# Autodesk Inventor assembly: 000 Ensamblaje hw_LM - BASIC
(part 2 of 3)
- Flush:121: RES-1.6K_1%_0402:40 ↔ RES-1.6K_1%_0402:43
- Mate:81: hw_LM - PCB:1 ↔ C1206C152KGRACAUTO:1
- Flush:122: C1206C152KGRACAUTO:3 ↔ C1206C152KGRACAUTO:4
- Flush:123: C1206C152KGRACAUTO:2 ↔ C1206C152KGRACAUTO:3
- Flush:124: C1206C152KGRACAUTO:1 ↔ C1206C152KGRACAUTO:2
- Flush:125: BLM21PG220SN1D:12 ↔ BLM21PG220SN1D:13
- Flush:126: BLM21PG220SN1D:13 ↔ BLM21PG220SN1D:14
- Flush:127: BLM21PG220SN1D:14 ↔ BLM21PG220SN1D:15
- [Flush]: AQ24CANFD-02HTG:6 ↔ AQ24CANFD-02HTG:7
- [Flush]: AQ24CANFD-02HTG:7 ↔ AQ24CANFD-02HTG:8
- [Flush]: AQ24CANFD-02HTG:5 ↔ AQ24CANFD-02HTG:8
- Mate:83: hw_LM - PCB:1 ↔ HX5008NL:3
- Flush:137: RES-1.6K_1%_0402:55 ↔ RES-1.6K_1%_0402:59
- Flush:138: RES-1.6K_1%_0402:44 ↔ RES-1.6K_1%_0402:56
- Flush:139: RES-1.6K_1%_0402:52 ↔ RES-1.6K_1%_0402:59
- Flush:142: RES-1.6K_1%_0402:23 ↔ RES-1.6K_1%_0402:47
- Mate:84: hw_LM - PCB:1 ↔ RES-1.6K_1%_0402:56
- Flush:143: RES-1.6K_1%_0402:48 ↔ RES-1.6K_1%_0402:57
- Flush:144: RES-1.6K_1%_0402:56 ↔ RES-1.6K_1%_0402:57
- Flush:145: RES-1.6K_1%_0402:55 ↔ RES-1.6K_1%_0402:59
- Flush:146: RES-1.6K_1%_0402:56 ↔ RES-1.6K_1%_0402:58
- Flush:147: RES-1.6K_1%_0402:55 ↔ RES-1.6K_1%_0402:59
- Flush:148: RES-1.6K_1%_0402:52 ↔ RES-1.6K_1%_0402:53
- Flush:149: RES-1.6K_1%_0402:54 ↔ RES-1.6K_1%_0402:55
- Flush:150: RES-1.6K_1%_0402:55 ↔ RES-1.6K_1%_0402:59
- Flush:151: RES-1.6K_1%_0402:56 ↔ RES-1.6K_1%_0402:59
- Flush:152: RES-1.6K_1%_0402:49 ↔ RES-1.6K_1%_0402:52
- Flush:153: RES-1.6K_1%_0402:50 ↔ RES-1.6K_1%_0402:51
- Flush:154: RES-1.6K_1%_0402:51 ↔ RES-1.6K_1%_0402:55
- Flush:155: RES-1.6K_1%_0402:44 ↔ RES-1.6K_1%_0402:46
- Flush:156: RES-1.6K_1%_0402:45 ↔ RES-1.6K_1%_0402:55
- [Flush]: RES-1.6K_1%_0402:60 ↔ RES-1.6K_1%_0402:62
- Flush:158: RES-1.6K_1%_0402:47 ↔ RES-1.6K_1%_0402:63
- Flush:159: RES-1.6K_1%_0402:60 ↔ RES-1.6K_1%_0402:63
- Flush:160: RES-1.6K_1%_0402:61 ↔ RES-1.6K_1%_0402:63
- [Flush]: RES-1.6K_1%_0402:64 ↔ RES-1.6K_1%_0402:66
- [Flush]: RES-1.6K_1%_0402:64 ↔ RES-1.6K_1%_0402:67
- [Flush]: RES-1.6K_1%_0402:65 ↔ RES-1.6K_1%_0402:67
- Flush:164: RES-1.6K_1%_0402:62 ↔ RES-1.6K_1%_0402:65
- [Flush]: RES-1.6K_1%_0402:68 ↔ RES-1.6K_1%_0402:70
- [Flush]: RES-1.6K_1%_0402:68 ↔ RES-1.6K_1%_0402:71
- [Flush]: RES-1.6K_1%_0402:69 ↔ RES-1.6K_1%_0402:71
- Flush:168: RES-1.6K_1%_0402:62 ↔ RES-1.6K_1%_0402:69
- [Flush]: RES-1.6K_1%_0402:72 ↔ RES-1.6K_1%_0402:73
- [Flush]: RES-1.6K_1%_0402:72 ↔ RES-1.6K_1%_0402:73
- [Flush]: RES-1.6K_1%_0402:74 ↔ RES-1.6K_1%_0402:75
- [Flush]: RES-1.6K_1%_0402:74 ↔ RES-1.6K_1%_0402:75
- [Flush]: RES-1.6K_1%_0402:73 ↔ RES-1.6K_1%_0402:74
- Flush:174: RES-1.6K_1%_0402:72 ↔ RES-1.6K_1%_0402:75
- Flush:175: RES-1.6K_1%_0402:63 ↔ RES-1.6K_1%_0402:74
- [Flush]: RES-1.6K_1%_0402:76 ↔ RES-1.6K_1%_0402:77
- [Flush]: RES-1.6K_1%_0402:76 ↔ RES-1.6K_1%_0402:77
- [Flush]: RES-1.6K_1%_0402:78 ↔ RES-1.6K_1%_0402:79
- [Flush]: RES-1.6K_1%_0402:78 ↔ RES-1.6K_1%_0402:79
- [Flush]: RES-1.6K_1%_0402:77 ↔ RES-1.6K_1%_0402:78
- [Flush]: RES-1.6K_1%_0402:76 ↔ RES-1.6K_1%_0402:79
- Flush:182: RES-1.6K_1%_0402:67 ↔ RES-1.6K_1%_0402:79
- Flush:183: RES-1.6K_1%_0402:66 ↔ RES-1.6K_1%_0402:76
- [Flush]: RES-1.6K_1%_0402:80 ↔ RES-1.6K_1%_0402:81
- [Flush]: RES-1.6K_1%_0402:80 ↔ RES-1.6K_1%_0402:81
- Flush:186: RES-1.6K_1%_0402:78 ↔ RES-1.6K_1%_0402:80
- [Flush]: RES-1.6K_1%_0402:82 ↔ RES-1.6K_1%_0402:83
- [Flush]: RES-1.6K_1%_0402:82 ↔ RES-1.6K_1%_0402:84
- [Flush]: RES-1.6K_1%_0402:84 ↔ RES-1.6K_1%_0402:85
- Flush:190: RES-1.6K_1%_0402:82 ↔ RES-1.6K_1%_0402:83
- Flush:191: RES-1.6K_1%_0402:83 ↔ RES-1.6K_1%_0402:84
- Flush:192: RES-1.6K_1%_0402:84 ↔ RES-1.6K_1%_0402:85
- Flush:194: RES-1.6K_1%_0402:85 ↔ RES-1.6K_1%_0402:86
- [Flush]: RES-1.6K_1%_0402:87 ↔ RES-1.6K_1%_0402:88
- [Flush]: RES-1.6K_1%_0402:87 ↔ RES-1.6K_1%_0402:88
- Flush:197: RES-1.6K_1%_0402:87 ↔ RES-1.6K_1%_0402:88
- Flush:198: RES-1.6K_1%_0402:30 ↔ RES-1.6K_1%_0402:87
- Mate:94: hw_LM - PCB:1 ↔ S32E288ABCAAMJGT:1
- Mate:95: hw_LM - PCB:1 ↔ DP83867ERGZT:1
- Mate:96: hw_LM - PCB:1 ↔ ECS-2520MVQ-250-CN-TR:2
- Angle:43 (0 deg): DP83867ERGZT:1 ↔ ECS-2520MVQ-250-CN-TR:2
- Mate:97: hw_LM - PCB:1 ↔ LTC7103IUHE#PBF:1
- Mate:98: hw_LM - PCB:1 ↔ TCAN1462VDRBRQ1:1
- Flush:200: TCAN1462VDRBRQ1:2 ↔ TCAN1462VDRBRQ1:3
- Flush:201: TCAN1462VDRBRQ1:1 ↔ TCAN1462VDRBRQ1:3
- Angle:44 (180 deg): hw_LM - PCB:1 ↔ HX5008NL:4
- Mate:99: hw_LM - PCB:1 ↔ HX5008NL:4
- Mate:100: hw_LM - PCB:1 ↔ SQJ465EP-T1_GE3:1
- Mate:101: hw_LM - PCB:1 ↔ SQJ465EP-T1_GE3:1
- Mate:102: hw_LM - PCB:1 ↔ KAM55CR72A106KV-C2220K-simpl:1
- Angle:45 (0 deg): hw_LM - PCB:1 ↔ KAM55CR72A106KV-C2220K-simpl:1
- Mate:103: hw_LM - PCB:1 ↔ KAM55CR72A106KV-C2220K-simpl:2
- Mate:104: hw_LM - PCB:1 ↔ STPS5H100AFY:1
- Angle:46 (0 deg): KAM55CR72A106KV-C2220K-simpl:1 ↔ STPS5H100AFY:1
- Mate:105: hw_LM - PCB:1 ↔ STPS5H100AFY:3
- Mate:107: hw_LM - PCB:1 ↔ SML-D12V8WT86C:2
- Mate:108: hw_LM - PCB:1 ↔ SML-D12V8WT86C:3
- Mate:109: hw_LM - PCB:1 ↔ SML-D12V8WT86C:4
- Mate:110: hw_LM - PCB:1 ↔ SML-D12V8WT86C:5
- Mate:112: hw_LM - PCB:1 ↔ RES-1.6K_1%_0402:92
- Mate:113: hw_LM - PCB:1 ↔ RES-1.6K_1%_0402:91
- Mate:114: hw_LM - PCB:1 ↔ RES-1.6K_1%_0402:90
- Mate:115: hw_LM - PCB:1 ↔ RES-1.6K_1%_0402:89
- Flush:202: SML-D12V8WT86C:2 ↔ SML-D12V8WT86C:6
- Flush:204: RES-1.6K_1%_0402:89 ↔ RES-1.6K_1%_0402:94
- Flush:205: RES-1.6K_1%_0402:89 ↔ RES-1.6K_1%_0402:90
- Flush:206: RES-1.6K_1%_0402:90 ↔ RES-1.6K_1%_0402:91
- Flush:207: RES-1.6K_1%_0402:91 ↔ RES-1.6K_1%_0402:92
- [Flush]: RES-1.6K_1%_0402:95 ↔ RES-1.6K_1%_0402:97
- [Flush]: RES-1.6K_1%_0402:95 ↔ RES-1.6K_1%_0402:96
- Mate:116: hw_LM - PCB:1 ↔ SMA6J64CA:1
- Angle:47 (0 deg): KAM55CR72A106KV-C2220K-simpl:1 ↔ SMA6J64CA:1
- Mate:117: hw_LM - PCB:1 ↔ SMA6J64CA:2
- Mate:118: hw_LM - PCB:1 ↔ C1210C472KGRACAUTO:1
- Flush:210: C1210C472KGRACAUTO:2 ↔ C1210C472KGRACAUTO:3
- Flush:211: C1210C472KGRACAUTO:1 ↔ C1210C472KGRACAUTO:2
- Angle:48 (0 deg): C1206C152KGRACAUTO:2 ↔ C1206C152KGRACAUTO:4
- Angle:49 (0 deg): hw_LM - PCB:1 ↔ C1206C152KGRACAUTO:1
- Angle:50 (0 deg): hw_LM - PCB:1 ↔ BSS123NH6327XTSA1:1
- Mate:119: hw_LM - PCB:1 ↔ BSS123NH6327XTSA1:1
- Mate:120: hw_LM - PCB:1 ↔ BZD27C10P-HE3-08:1
- Mate:121: hw_LM - PCB:1 ↔ C0603C103K1RECAUTO:1
- Flush:212: C0603C103K1RECAUTO:5 ↔ C0603C103K1RECAUTO:6
- Flush:213: C0603C103K1RECAUTO:2 ↔ C0603C103K1RECAUTO:5
- Flush:214: C0603C103K1RECAUTO:2 ↔ C0603C103K1RECAUTO:7
- Flush:215: C0603C103K1RECAUTO:4 ↔ C0603C103K1RECAUTO:6
- Flush:216: C0603C103K1RECAUTO:5 ↔ C0603C103K1RECAUTO:8
- Flush:217: C0603C103K1RECAUTO:1 ↔ C0603C103K1RECAUTO:5
- Flush:218: C0603C103K1RECAUTO:3 ↔ C0603C103K1RECAUTO:8
- Flush:219: C0603C103K1RECAUTO:1 ↔ C0603C103K1RECAUTO:8
- [Flush]: C0603C103K1RECAUTO:9 ↔ C0603C103K1RECAUTO:11
- Angle:53 (0 deg): hw_LM - PCB:1 ↔ C0603C103K1RECAUTO:9
- Flush:221: C1206C152KGRACAUTO:3 ↔ C0603C103K1RECAUTO:10
- Flush:222: C1206C152KGRACAUTO:3 ↔ C0603C103K1RECAUTO:9
- Flush:223: C0603C103K1RECAUTO:9 ↔ C0603C103K1RECAUTO:11
- Flush:224: C1210C472KGRACAUTO:7 ↔ C1210C472KGRACAUTO:8
- Mate:122: hw_LM - PCB:1 ↔ LM5146QRGYRQ1:1
- Mate:123: hw_LM - PCB:1 ↔ 1812CAN-113NRC:1
- Mate:124: hw_LM - PCB:1 ↔ TCAN1462VDRBRQ1:5
- Flush:228: C1210C472KGRACAUTO:11 ↔ C1210C472KGRACAUTO:12
- Flush:229: C1210C472KGRACAUTO:9 ↔ C1210C472KGRACAUTO:10
- Flush:230: C1210C472KGRACAUTO:11 ↔ C1210C472KGRACAUTO:12
- Flush:231: C1210C472KGRACAUTO:8 ↔ C1210C472KGRACAUTO:9
- Flush:232: C1210C472KGRACAUTO:11 ↔ C1210C472KGRACAUTO:12
- [Flush]: RES-1.6K_1%_0402:98 ↔ RES-1.6K_1%_0402:99
- [Flush]: RES-1.6K_1%_0402:98 ↔ RES-1.6K_1%_0402:99
- [Flush]: RES-1.6K_1%_0402:100 ↔ RES-1.6K_1%_0402:101
- [Flush]: RES-1.6K_1%_0402:100 ↔ RES-1.6K_1%_0402:101
- [Flush]: RES-1.6K_1%_0402:102 ↔ RES-1.6K_1%_0402:103
- [Flush]: RES-1.6K_1%_0402:102 ↔ RES-1.6K_1%_0402:103
- Flush:240: RES-1.6K_1%_0402:100 ↔ RES-1.6K_1%_0402:102
- Flush:241: RES-1.6K_1%_0402:101 ↔ RES-1.6K_1%_0402:103
- Flush:242: RES-1.6K_1%_0402:98 ↔ RES-1.6K_1%_0402:99
- Flush:243: RES-1.6K_1%_0402:99 ↔ RES-1.6K_1%_0402:100
- Flush:244: RES-1.6K_1%_0402:101 ↔ RES-1.6K_1%_0402:103
- Flush:245: RES-1.6K_1%_0402:9 ↔ RES-1.6K_1%_0402:98
- Flush:246: RES-1.6K_1%_0402:85 ↔ RES-1.6K_1%_0402:102
- Mate:125: hw_LM - PCB:1 ↔ RES-1.6K_1%_0402:100
- [Flush]: RES-1.6K_1%_0402:105 ↔ RES-1.6K_1%_0402:106
- [Flush]: RES-1.6K_1%_0402:108 ↔ RES-1.6K_1%_0402:109
- Flush:249: RES-1.6K_1%_0402:107 ↔ RES-1.6K_1%_0402:109
- Flush:250: RES-1.6K_1%_0402:106 ↔ RES-1.6K_1%_0402:108
- Flush:251: RES-1.6K_1%_0402:104 ↔ RES-1.6K_1%_0402:109
- Flush:252: RES-1.6K_1%_0402:105 ↔ RES-1.6K_1%_0402:107
- Flush:253: RES-1.6K_1%_0402:9 ↔ RES-1.6K_1%_0402:106
- [Flush]: RES-1.6K_1%_0402:111 ↔ RES-1.6K_1%_0402:112
- [Flush]: RES-1.6K_1%_0402:114 ↔ RES-1.6K_1%_0402:115
- [Flush]: RES-1.6K_1%_0402:113 ↔ RES-1.6K_1%_0402:115
- [Flush]: RES-1.6K_1%_0402:112 ↔ RES-1.6K_1%_0402:114
- [Flush]: RES-1.6K_1%_0402:110 ↔ RES-1.6K_1%_0402:115
- [Flush]: RES-1.6K_1%_0402:111 ↔ RES-1.6K_1%_0402:113
- Flush:260: RES-1.6K_1%_0402:107 ↔ RES-1.6K_1%_0402:112
- Flush:261: RES-1.6K_1%_0402:105 ↔ RES-1.6K_1%_0402:113
- [Flush]: RES-1.6K_1%_0402:117 ↔ RES-1.6K_1%_0402:118
- [Flush]: RES-1.6K_1%_0402:120 ↔ RES-1.6K_1%_0402:121
- [Flush]: RES-1.6K_1%_0402:119 ↔ RES-1.6K_1%_0402:121
- [Flush]: RES-1.6K_1%_0402:118 ↔ RES-1.6K_1%_0402:120
- [Flush]: RES-1.6K_1%_0402:116 ↔ RES-1.6K_1%_0402:121
- [Flush]: RES-1.6K_1%_0402:117 ↔ RES-1.6K_1%_0402:119
- [Flush]: RES-1.6K_1%_0402:123 ↔ RES-1.6K_1%_0402:124
- [Flush]: RES-1.6K_1%_0402:126 ↔ RES-1.6K_1%_0402:127
- [Flush]: RES-1.6K_1%_0402:125 ↔ RES-1.6K_1%_0402:127
- [Flush]: RES-1.6K_1%_0402:124 ↔ RES-1.6K_1%_0402:126
- [Flush]: RES-1.6K_1%_0402:122 ↔ RES-1.6K_1%_0402:127
- [Flush]: RES-1.6K_1%_0402:123 ↔ RES-1.6K_1%_0402:125
- [Flush]: RES-1.6K_1%_0402:119 ↔ RES-1.6K_1%_0402:124
- [Flush]: RES-1.6K_1%_0402:117 ↔ RES-1.6K_1%_0402:125
- Flush:276: RES-1.6K_1%_0402:115 ↔ RES-1.6K_1%_0402:122
- Flush:277: RES-1.6K_1%_0402:120 ↔ RES-1.6K_1%_0402:126
- Flush:278: RES-1.6K_1%_0402:105 ↔ RES-1.6K_1%_0402:120
- [Flush]: RES-1.6K_1%_0402:129 ↔ RES-1.6K_1%_0402:130
- [Flush]: RES-1.6K_1%_0402:132 ↔ RES-1.6K_1%_0402:133
- [Flush]: RES-1.6K_1%_0402:131 ↔ RES-1.6K_1%_0402:133
- [Flush]: RES-1.6K_1%_0402:130 ↔ RES-1.6K_1%_0402:132
- [Flush]: RES-1.6K_1%_0402:128 ↔ RES-1.6K_1%_0402:133
- [Flush]: RES-1.6K_1%_0402:129 ↔ RES-1.6K_1%_0402:131
- [Flush]: RES-1.6K_1%_0402:135 ↔ RES-1.6K_1%_0402:136
- [Flush]: RES-1.6K_1%_0402:138 ↔ RES-1.6K_1%_0402:139
- [Flush]: RES-1.6K_1%_0402:137 ↔ RES-1.6K_1%_0402:139
- [Flush]: RES-1.6K_1%_0402:136 ↔ RES-1.6K_1%_0402:138
- [Flush]: RES-1.6K_1%_0402:134 ↔ RES-1.6K_1%_0402:139
- [Flush]: RES-1.6K_1%_0402:135 ↔ RES-1.6K_1%_0402:137
- [Flush]: RES-1.6K_1%_0402:131 ↔ RES-1.6K_1%_0402:136
- [Flush]: RES-1.6K_1%_0402:129 ↔ RES-1.6K_1%_0402:137
- [Flush]: RES-1.6K_1%_0402:132 ↔ RES-1.6K_1%_0402:138
- Flush:294: RES-1.6K_1%_0402:134 ↔ RES-1.6K_1%_0402:139
- Flush:295: RES-1.6K_1%_0402:117 ↔ RES-1.6K_1%_0402:139
- Flush:296: RES-1.6K_1%_0402:113 ↔ RES-1.6K_1%_0402:137
- [Flush]: RES-1.6K_1%_0402:140 ↔ RES-1.6K_1%_0402:141
- [Flush]: RES-1.6K_1%_0402:144 ↔ RES-1.6K_1%_0402:145
- [Flush]: RES-1.6K_1%_0402:143 ↔ RES-1.6K_1%_0402:145
- [Flush]: RES-1.6K_1%_0402:142 ↔ RES-1.6K_1%_0402:145
- [Flush]: RES-1.6K_1%_0402:148 ↔ RES-1.6K_1%_0402:149
- [Flush]: RES-1.6K_1%_0402:147 ↔ RES-1.6K_1%_0402:149
- [Flush]: RES-1.6K_1%_0402:146 ↔ RES-1.6K_1%_0402:149
- [Flush]: RES-1.6K_1%_0402:144 ↔ RES-1.6K_1%_0402:148
- [Flush]: RES-1.6K_1%_0402:146 ↔ RES-1.6K_1%_0402:149
- [Flush]: RES-1.6K_1%_0402:140 ↔ RES-1.6K_1%_0402:149
- [Flush]: RES-1.6K_1%_0402:150 ↔ RES-1.6K_1%_0402:151
- [Flush]: RES-1.6K_1%_0402:154 ↔ RES-1.6K_1%_0402:155
- [Flush]: RES-1.6K_1%_0402:153 ↔ RES-1.6K_1%_0402:155
- [Flush]: RES-1.6K_1%_0402:152 ↔ RES-1.6K_1%_0402:155
- [Flush]: RES-1.6K_1%_0402:158 ↔ RES-1.6K_1%_0402:159
- [Flush]: RES-1.6K_1%_0402:157 ↔ RES-1.6K_1%_0402:159
- [Flush]: RES-1.6K_1%_0402:156 ↔ RES-1.6K_1%_0402:159
- [Flush]: RES-1.6K_1%_0402:154 ↔ RES-1.6K_1%_0402:158
- [Flush]: RES-1.6K_1%_0402:156 ↔ RES-1.6K_1%_0402:159
- [Flush]: RES-1.6K_1%_0402:150 ↔ RES-1.6K_1%_0402:159
- Flush:317: RES-1.6K_1%_0402:145 ↔ RES-1.6K_1%_0402:157
- Flush:318: RES-1.6K_1%_0402:147 ↔ RES-1.6K_1%_0402:155
- Flush:319: RES-1.6K_1%_0402:113 ↔ RES-1.6K_1%_0402:150
- [Flush]: RES-1.6K_1%_0402:162 ↔ RES-1.6K_1%_0402:163
- [Flush]: RES-1.6K_1%_0402:161 ↔ RES-1.6K_1%_0402:163
- [Flush]: RES-1.6K_1%_0402:160 ↔ RES-1.6K_1%_0402:163
- Flush:323: RES-1.6K_1%_0402:145 ↔ RES-1.6K_1%_0402:163
- Flush:324: RES-1.6K_1%_0402:144 ↔ RES-1.6K_1%_0402:161
- Flush:325: RES-1.6K_1%_0402:161 ↔ RES-1.6K_1%_0402:162
- Flush:326: RES-1.6K_1%_0402:146 ↔ RES-1.6K_1%_0402:160
- Flush:327: RES-1.6K_1%_0402:143 ↔ RES-1.6K_1%_0402:164
- Flush:328: RES-1.6K_1%_0402:145 ↔ RES-1.6K_1%_0402:161
- Flush:329: RES-1.6K_1%_0402:100 ↔ RES-1.6K_1%_0402:142
- Mate:126: hw_LM - PCB:1 ↔ HSP051-4M10:1
- Flush:330: HSP051-4M10:1 ↔ HSP051-4M10:2
- Angle:56 (0 deg): C0603C101K5GAC3190:6 ↔ C0603C101K5GAC3190:7
- Mate:127 (0.75 mm): hw_LM - PCB:1 ↔ ADIS16505-3BMLZ:1
- Mate:128: hw_LM - PCB:1 ↔ BMI088:2
- Mate:129: hw_LM - PCB:1 ↔ ESIM 638037665970:1
- Angle:58 (0 deg): S32E288ABCAAMJGT:1 ↔ ESIM 638037665970:1
- Mate:130: hw_LM - PCB:1 ↔ TPS7A5301QRGRRQ1:2
- Mate:131: hw_LM - PCB:1 ↔ LTC2875MPDD#PBF:1
- Mate:132: hw_LM - PCB:1 ↔ UQFN-16:1
- Angle:59 (0 deg): hw_LM - PCB:1 ↔ UQFN-16:1
- Flush:331: LTC2875MPDD#PBF:1 ↔ LTC2875MPDD#PBF:2
- Mate:133: hw_LM - PCB:1 ↔ ECS-400-8-33Q-ADS-TR:1
- Angle:60 (0 deg): S32E288ABCAAMJGT:1 ↔ ECS-400-8-33Q-ADS-TR:1
- Mate:134: hw_LM - PCB:1 ↔ TPS3897ADRYT:1
- Flush:332: HSP051-4M10:1 ↔ HSP051-4M10:3
- Angle:62 (180 deg): hw_LM - PCB:1 ↔ PESD2CANFD27V-UX:1
- Mate:135: hw_LM - PCB:1 ↔ PESD2CANFD27V-UX:1
- Angle:63 (0 deg): SMA6J64CA:1 ↔ PESD2CANFD27V-UX:1
- Angle:64 (180 deg): hw_LM - PCB:1 ↔ DMN2710UTQ-7:1
- Mate:136: hw_LM - PCB:1 ↔ DMN2710UTQ-7:1
- Angle:65 (180 deg): C1210C472KGRACAUTO:12 ↔ DMN2710UTQ-7:1
- Flush:333: DMN2710UTQ-7:1 ↔ DMN2710UTQ-7:2
- Flush:334: C0603C103K1RECAUTO:12 ↔ C0603C103K1RECAUTO:13
- Flush:335: C0603C103K1RECAUTO:1 ↔ C0603C103K1RECAUTO:13
- Flush:336: C0603C103K1RECAUTO:14 ↔ C0603C103K1RECAUTO:15
- Flush:337: C0603C103K1RECAUTO:6 ↔ C0603C103K1RECAUTO:14
- Flush:338: DMN2710UTQ-7:2 ↔ DMN2710UTQ-7:4
- Flush:339: DMN2710UTQ-7:3 ↔ DMN2710UTQ-7:4
- Flush:340: DMN2710UTQ-7:3 ↔ DMN2710UTQ-7:5
- [Flush]: RES-1.6K_1%_0402:167 ↔ RES-1.6K_1%_0402:168
- [Flush]: RES-1.6K_1%_0402:166 ↔ RES-1.6K_1%_0402:168
- [Flush]: RES-1.6K_1%_0402:165 ↔ RES-1.6K_1%_0402:168
- Flush:344: RES-1.6K_1%_0402:142 ↔ RES-1.6K_1%_0402:167
- Flush:345: RES-1.6K_1%_0402:143 ↔ RES-1.6K_1%_0402:165
- Flush:346: RES-1.6K_1%_0402:146 ↔ RES-1.6K_1%_0402:168
- [Flush]: RES-1.6K_1%_0402:175 ↔ RES-1.6K_1%_0402:176
- [Flush]: RES-1.6K_1%_0402:174 ↔ RES-1.6K_1%_0402:176
- [Flush]: RES-1.6K_1%_0402:173 ↔ RES-1.6K_1%_0402:176
- [Flush]: RES-1.6K_1%_0402:170 ↔ RES-1.6K_1%_0402:175
- [Flush]: RES-1.6K_1%_0402:171 ↔ RES-1.6K_1%_0402:173
- [Flush]: RES-1.6K_1%_0402:172 ↔ RES-1.6K_1%_0402:176
- Flush:353: RES-1.6K_1%_0402:143 ↔ RES-1.6K_1%_0402:177
- Flush:354: RES-1.6K_1%_0402:146 ↔ RES-1.6K_1%_0402:175
- Flush:355: RES-1.6K_1%_0402:170 ↔ RES-1.6K_1%_0402:176
- Flush:356: RES-1.6K_1%_0402:171 ↔ RES-1.6K_1%_0402:177
- [Flush]: RES-1.6K_1%_0402:183 ↔ RES-1.6K_1%_0402:184
- [Flush]: RES-1.6K_1%_0402:182 ↔ RES-1.6K_1%_0402:184
- [Flush]: RES-1.6K_1%_0402:181 ↔ RES-1.6K_1%_0402:184
- [Flush]: RES-1.6K_1%_0402:178 ↔ RES-1.6K_1%_0402:183
- [Flush]: RES-1.6K_1%_0402:179 ↔ RES-1.6K_1%_0402:181
- [Flush]: RES-1.6K_1%_0402:180 ↔ RES-1.6K_1%_0402:184
- [Flush]: RES-1.6K_1%_0402:178 ↔ RES-1.6K_1%_0402:184
- [Flush]: RES-1.6K_1%_0402:179 ↔ RES-1.6K_1%_0402:185
- [Flush]: RES-1.6K_1%_0402:191 ↔ RES-1.6K_1%_0402:192
- [Flush]: RES-1.6K_1%_0402:190 ↔ RES-1.6K_1%_0402:192
- [Flush]: RES-1.6K_1%_0402:189 ↔ RES-1.6K_1%_0402:192
- [Flush]: RES-1.6K_1%_0402:186 ↔ RES-1.6K_1%_0402:191
- [Flush]: RES-1.6K_1%_0402:187 ↔ RES-1.6K_1%_0402:189
- [Flush]: RES-1.6K_1%_0402:188 ↔ RES-1.6K_1%_0402:192
- [Flush]: RES-1.6K_1%_0402:186 ↔ RES-1.6K_1%_0402:192
- [Flush]: RES-1.6K_1%_0402:187 ↔ RES-1.6K_1%_0402:193
- [Flush]: RES-1.6K_1%_0402:199 ↔ RES-1.6K_1%_0402:200
- [Flush]: RES-1.6K_1%_0402:198 ↔ RES-1.6K_1%_0402:200
- [Flush]: RES-1.6K_1%_0402:197 ↔ RES-1.6K_1%_0402:200
- [Flush]: RES-1.6K_1%_0402:194 ↔ RES-1.6K_1%_0402:199
- [Flush]: RES-1.6K_1%_0402:195 ↔ RES-1.6K_1%_0402:197
- [Flush]: RES-1.6K_1%_0402:196 ↔ RES-1.6K_1%_0402:200
- [Flush]: RES-1.6K_1%_0402:194 ↔ RES-1.6K_1%_0402:200
- [Flush]: RES-1.6K_1%_0402:195 ↔ RES-1.6K_1%_0402:201
- Flush:381: RES-1.6K_1%_0402:174 ↔ RES-1.6K_1%_0402:182
- Flush:382: RES-1.6K_1%_0402:170 ↔ RES-1.6K_1%_0402:183
- Flush:383: RES-1.6K_1%_0402:183 ↔ RES-1.6K_1%_0402:198
- Flush:384: RES-1.6K_1%_0402:185 ↔ RES-1.6K_1%_0402:200
- Flush:385: RES-1.6K_1%_0402:190 ↔ RES-1.6K_1%_0402:199
- Flush:386: RES-1.6K_1%_0402:187 ↔ RES-1.6K_1%_0402:197
- Flush:387: RES-1.6K_1%_0402:188 ↔ RES-1.6K_1%_0402:201
- Flush:388: RES-1.6K_1%_0402:189 ↔ RES-1.6K_1%_0402:200
- Angle:69 (0 deg): RES-1.6K_1%_0402:191 ↔ RES-1.6K_1%_0402:192
- Angle:70 (0 deg): RES-1.6K_1%_0402:190 ↔ RES-1.6K_1%_0402:191
- Angle:71 (0 deg): RES-1.6K_1%_0402:189 ↔ RES-1.6K_1%_0402:190
- Angle:72 (0 deg): RES-1.6K_1%_0402:189 ↔ RES-1.6K_1%_0402:193
- Angle:73 (0 deg): RES-1.6K_1%_0402:186 ↔ RES-1.6K_1%_0402:193
- Angle:74 (0 deg): RES-1.6K_1%_0402:186 ↔ RES-1.6K_1%_0402:187
- Angle:75 (0 deg): RES-1.6K_1%_0402:188 ↔ RES-1.6K_1%_0402:189
- Angle:76 (0 deg): LM5146QRGYRQ1:1 ↔ RES-1.6K_1%_0402:192
- [Flush]: RES-1.6K_1%_0402:207 ↔ RES-1.6K_1%_0402:208
- [Flush]: RES-1.6K_1%_0402:206 ↔ RES-1.6K_1%_0402:208
- [Flush]: RES-1.6K_1%_0402:205 ↔ RES-1.6K_1%_0402:208
- [Flush]: RES-1.6K_1%_0402:202 ↔ RES-1.6K_1%_0402:207
- [Flush]: RES-1.6K_1%_0402:203 ↔ RES-1.6K_1%_0402:205
- [Flush]: RES-1.6K_1%_0402:204 ↔ RES-1.6K_1%_0402:208
- [Flush]: RES-1.6K_1%_0402:202 ↔ RES-1.6K_1%_0402:208
- [Flush]: RES-1.6K_1%_0402:203 ↔ RES-1.6K_1%_0402:209
- [Angle] (0 deg): RES-1.6K_1%_0402:207 ↔ RES-1.6K_1%_0402:208
- [Angle] (0 deg): RES-1.6K_1%_0402:206 ↔ RES-1.6K_1%_0402:207
- [Angle] (0 deg): RES-1.6K_1%_0402:205 ↔ RES-1.6K_1%_0402:206
- [Angle] (0 deg): RES-1.6K_1%_0402:205 ↔ RES-1.6K_1%_0402:209
- [Angle] (0 deg): RES-1.6K_1%_0402:202 ↔ RES-1.6K_1%_0402:209
- [Angle] (0 deg): RES-1.6K_1%_0402:202 ↔ RES-1.6K_1%_0402:203
- [Angle] (0 deg): RES-1.6K_1%_0402:204 ↔ RES-1.6K_1%_0402:205
- Flush:397: RES-1.6K_1%_0402:193 ↔ RES-1.6K_1%_0402:204
- Flush:398: RES-1.6K_1%_0402:191 ↔ RES-1.6K_1%_0402:202
- Flush:399: RES-1.6K_1%_0402:186 ↔ RES-1.6K_1%_0402:206
- [Flush]: RES-1.6K_1%_0402:212 ↔ RES-1.6K_1%_0402:213
- [Flush]: RES-1.6K_1%_0402:212 ↔ RES-1.6K_1%_0402:213
- [Flush]: RES-1.6K_1%_0402:211 ↔ RES-1.6K_1%_0402:213
- [Flush]: RES-1.6K_1%_0402:211 ↔ RES-1.6K_1%_0402:213
- [Flush]: RES-1.6K_1%_0402:215 ↔ RES-1.6K_1%_0402:216
- [Flush]: RES-1.6K_1%_0402:214 ↔ RES-1.6K_1%_0402:216
- [Flush]: RES-1.6K_1%_0402:219 ↔ RES-1.6K_1%_0402:220
- [Flush]: RES-1.6K_1%_0402:219 ↔ RES-1.6K_1%_0402:220
- [Flush]: RES-1.6K_1%_0402:218 ↔ RES-1.6K_1%_0402:220
- [Flush]: RES-1.6K_1%_0402:218 ↔ RES-1.6K_1%_0402:220
- [Flush]: RES-1.6K_1%_0402:222 ↔ RES-1.6K_1%_0402:223
- [Flush]: RES-1.6K_1%_0402:221 ↔ RES-1.6K_1%_0402:223
- Flush:412: RES-1.6K_1%_0402:215 ↔ RES-1.6K_1%_0402:220
- Flush:413: RES-1.6K_1%_0402:210 ↔ RES-1.6K_1%_0402:219
- Flush:414: RES-1.6K_1%_0402:216 ↔ RES-1.6K_1%_0402:217
- Flush:415: RES-1.6K_1%_0402:220 ↔ RES-1.6K_1%_0402:222
- Flush:416: RES-1.6K_1%_0402:213 ↔ RES-1.6K_1%_0402:223
- Flush:417: RES-1.6K_1%_0402:215 ↔ RES-1.6K_1%_0402:221
- Flush:418: RES-1.6K_1%_0402:214 ↔ RES-1.6K_1%_0402:217
- Flush:419: RES-1.6K_1%_0402:210 ↔ RES-1.6K_1%_0402:217
- Flush:420: RES-1.6K_1%_0402:31 ↔ RES-1.6K_1%_0402:220
- [Flush]: DMN2710UTQ-7:6 ↔ DMN2710UTQ-7:7
- Flush:422: DMN2710UTQ-7:4 ↔ DMN2710UTQ-7:7
- Flush:423: DMN2710UTQ-7:7 ↔ DMN2710UTQ-7:8
- Angle:86 (180 deg): hw_LM - PCB:1 ↔ SN74LVC1G08QDCKRQ1:1
- Mate:137: hw_LM - PCB:1 ↔ SN74LVC1G08QDCKRQ1:1
- Flush:424: C0603C103K1RECAUTO:16 ↔ C0603C103K1RECAUTO:18
- Flush:425: C0603C103K1RECAUTO:17 ↔ C0603C103K1RECAUTO:19
- Flush:426: C0603C103K1RECAUTO:16 ↔ C0603C103K1RECAUTO:17
- Flush:427: C0603C103K1RECAUTO:7 ↔ C0603C103K1RECAUTO:16
- [Flush]: C0603C103K1RECAUTO:20 ↔ C0603C103K1RECAUTO:22
- [Flush]: C0603C103K1RECAUTO:21 ↔ C0603C103K1RECAUTO:23
- [Flush]: C0603C103K1RECAUTO:20 ↔ C0603C103K1RECAUTO:21
- Flush:431: C0603C103K1RECAUTO:17 ↔ C0603C103K1RECAUTO:21
- Mate:138: hw_LM - PCB:1 ↔ UQFN-16:2
- Flush:432: C1206C152KGRACAUTO:3 ↔ C1206C152KGRACAUTO:5
- Mate:139: hw_LM - PCB:1 ↔ RES-1.6K_1%_0402:97
- Mate:140: hw_LM - PCB:1 ↔ 53398-0471:1
- Angle:88 (180 deg): hw_LM - PCB:1 ↔ 53398-0471:1
- Mate:141: hw_LM - PCB:1 ↔ XAL7030-472MEC:1
- Flush:433: XAL7030-472MEC:1 ↔ XAL7030-472MEC:2
- Mate:142: hw_LM - PCB:1 ↔ SQJ402EP-T1_GE3:1
- Mate:143: hw_LM - PCB:1 ↔ SQJ402EP-T1_GE3:1
- Mate:144: hw_LM - PCB:1 ↔ SQJ402EP-T1_GE3:2
- Mate:145: hw_LM - PCB:1 ↔ SQJ402EP-T1_GE3:2
- Tangent:1: hw_LM - PCB:1 ↔ MMB02070B1007GB200:1
- Mate:146: hw_LM - PCB:1 ↔ C1210C472KGRACAUTO:13
- Mate:147: hw_LM - PCB:1 ↔ C1206C152KGRACAUTO:6
- Flush:436: C1206C152KGRACAUTO:7 ↔ C1206C152KGRACAUTO:8
- Mate:148: hw_LM - PCB:1 ↔ R0805:4
- Flush:437: R0805:4 ↔ R0805:7
- Flush:438: R0805:5 ↔ R0805:7
- Flush:439: R0805:5 ↔ R0805:6
- Flush:440: R0805:4 ↔ R0805:6
- [Flush]: R0805:8 ↔ R0805:10
- [Flush]: R0805:8 ↔ R0805:9
- Flush:443: R0805:4 ↔ R0805:10
- Mate:149: hw_LM - PCB:1 ↔ 1812CAN-113NRC:2
- Mate:150: hw_LM - PCB:1 ↔ XAL4020-601MEC:1
- Flush:444: XAL4020-601MEC:1 ↔ XAL4020-601MEC:2
- Mate:151: hw_LM - PCB:1 ↔ BZD27C10P-HE3-08:2
- Mate:152: hw_LM - PCB:1 ↔ LTC3310SIV#PBF:1
- Flush:446: LTC3310SIV#PBF:1 ↔ LTC3310SIV#PBF:2
- Mate:153: hw_LM - PCB:1 ↔ TPD4E05U06QDQARQ1:1
- Flush:447: TPD4E05U06QDQARQ1:1 ↔ TPD4E05U06QDQARQ1:3
- Flush:448: TPD4E05U06QDQARQ1:2 ↔ TPD4E05U06QDQARQ1:3
- Mate:154: hw_LM - PCB:1 ↔ P3767-pcba-envelop_20230310:1
- Mate:155: hw_LM - PCB:1 ↔ P3767-pcba-envelop_20230310:1
- Flush:450: RES-1.6K_1%_0402:226 ↔ RES-1.6K_1%_0402:227
- Flush:451: RES-1.6K_1%_0402:97 ↔ RES-1.6K_1%_0402:226
- Flush:452: RES-1.6K_1%_0402:224 ↔ RES-1.6K_1%_0402:226
- Flush:453: RES-1.6K_1%_0402:225 ↔ RES-1.6K_1%_0402:226
- Flush:454: RES-1.6K_1%_0402:225 ↔ RES-1.6K_1%_0402:227
- [Flush]: RES-1.6K_1%_0402:230 ↔ RES-1.6K_1%_0402:231
- [Flush]: RES-1.6K_1%_0402:228 ↔ RES-1.6K_1%_0402:230
- [Flush]: RES-1.6K_1%_0402:229 ↔ RES-1.6K_1%_0402:230
- [Flush]: RES-1.6K_1%_0402:229 ↔ RES-1.6K_1%_0402:231
- [Flush]: RES-1.6K_1%_0402:234 ↔ RES-1.6K_1%_0402:235
- [Flush]: RES-1.6K_1%_0402:232 ↔ RES-1.6K_1%_0402:234
- [Flush]: RES-1.6K_1%_0402:233 ↔ RES-1.6K_1%_0402:234
- [Flush]: RES-1.6K_1%_0402:233 ↔ RES-1.6K_1%_0402:235
- Flush:463: RES-1.6K_1%_0402:225 ↔ RES-1.6K_1%_0402:230
- Flush:464: RES-1.6K_1%_0402:229 ↔ RES-1.6K_1%_0402:232
- Flush:465: RES-1.6K_1%_0402:228 ↔ RES-1.6K_1%_0402:233
- Flush:466: RES-1.6K_1%_0402:224 ↔ RES-1.6K_1%_0402:235
- Flush:467: RES-1.6K_1%_0402:97 ↔ RES-1.6K_1%_0402:226
- [Flush]: RES-1.6K_1%_0402:238 ↔ RES-1.6K_1%_0402:239
- [Flush]: RES-1.6K_1%_0402:236 ↔ RES-1.6K_1%_0402:238
- [Flush]: RES-1.6K_1%_0402:237 ↔ RES-1.6K_1%_0402:238
- [Flush]: RES-1.6K_1%_0402:237 ↔ RES-1.6K_1%_0402:239
- [Flush]: RES-1.6K_1%_0402:242 ↔ RES-1.6K_1%_0402:243
- [Flush]: RES-1.6K_1%_0402:240 ↔ RES-1.6K_1%_0402:242
- [Flush]: RES-1.6K_1%_0402:241 ↔ RES-1.6K_1%_0402:242
- [Flush]: RES-1.6K_1%_0402:241 ↔ RES-1.6K_1%_0402:243
- Flush:476: RES-1.6K_1%_0402:226 ↔ RES-1.6K_1%_0402:239
- Flush:477: RES-1.6K_1%_0402:232 ↔ RES-1.6K_1%_0402:237
- Flush:478: RES-1.6K_1%_0402:236 ↔ RES-1.6K_1%_0402:241
- Flush:479: RES-1.6K_1%_0402:97 ↔ RES-1.6K_1%_0402:234
- Flush:480: RES-1.6K_1%_0402:234 ↔ RES-1.6K_1%_0402:240
- [Flush]: RES-1.6K_1%_0402:246 ↔ RES-1.6K_1%_0402:247
- [Flush]: RES-1.6K_1%_0402:244 ↔ RES-1.6K_1%_0402:246
- [Flush]: RES-1.6K_1%_0402:245 ↔ RES-1.6K_1%_0402:246
- [Flush]: RES-1.6K_1%_0402:245 ↔ RES-1.6K_1%_0402:247
- [Flush]: RES-1.6K_1%_0402:250 ↔ RES-1.6K_1%_0402:251
- [Flush]: RES-1.6K_1%_0402:248 ↔ RES-1.6K_1%_0402:250
- [Flush]: RES-1.6K_1%_0402:249 ↔ RES-1.6K_1%_0402:250
- [Flush]: RES-1.6K_1%_0402:249 ↔ RES-1.6K_1%_0402:251
- Flush:489: RES-1.6K_1%_0402:242 ↔ RES-1.6K_1%_0402:246
- Flush:490: RES-1.6K_1%_0402:246 ↔ RES-1.6K_1%_0402:248
- Flush:491: RES-1.6K_1%_0402:247 ↔ RES-1.6K_1%_0402:249
- Flush:492: RES-1.6K_1%_0402:97 ↔ RES-1.6K_1%_0402:249
- [Flush]: RES-1.6K_1%_0402:254 ↔ RES-1.6K_1%_0402:255
- [Flush]: RES-1.6K_1%_0402:252 ↔ RES-1.6K_1%_0402:254
- [Flush]: RES-1.6K_1%_0402:253 ↔ RES-1.6K_1%_0402:254
- [Flush]: RES-1.6K_1%_0402:253 ↔ RES-1.6K_1%_0402:255
- [Flush]: RES-1.6K_1%_0402:258 ↔ RES-1.6K_1%_0402:259
- [Flush]: RES-1.6K_1%_0402:256 ↔ RES-1.6K_1%_0402:258
- [Flush]: RES-1.6K_1%_0402:257 ↔ RES-1.6K_1%_0402:258
- [Flush]: RES-1.6K_1%_0402:257 ↔ RES-1.6K_1%_0402:259
- Flush:501: RES-1.6K_1%_0402:251 ↔ RES-1.6K_1%_0402:255
- Flush:502: RES-1.6K_1%_0402:253 ↔ RES-1.6K_1%_0402:259
- Flush:503: RES-1.6K_1%_0402:248 ↔ RES-1.6K_1%_0402:258
- Flush:504: RES-1.6K_1%_0402:253 ↔ RES-1.6K_1%_0402:256
- [Flush]: RES-1.6K_1%_0402:261 ↔ RES-1.6K_1%_0402:262
- [Flush]: RES-1.6K_1%_0402:260 ↔ RES-1.6K_1%_0402:261
- [Flush]: RES-1.6K_1%_0402:260 ↔ RES-1.6K_1%_0402:262
- [Flush]: RES-1.6K_1%_0402:264 ↔ RES-1.6K_1%_0402:265
- [Flush]: RES-1.6K_1%_0402:263 ↔ RES-1.6K_1%_0402:264
- [Flush]: RES-1.6K_1%_0402:263 ↔ RES-1.6K_1%_0402:265
- Angle:91 (0 deg): hw_LM - PCB:1 ↔ RES-1.6K_1%_0402:258
- Angle:92 (0 deg): RES-1.6K_1%_0402:258 ↔ RES-1.6K_1%_0402:259
- Angle:93 (0 deg): RES-1.6K_1%_0402:257 ↔ RES-1.6K_1%_0402:258
- Angle:94 (0 deg): RES-1.6K_1%_0402:257 ↔ RES-1.6K_1%_0402:264
- Angle:95 (0 deg): RES-1.6K_1%_0402:263 ↔ RES-1.6K_1%_0402:264
- Angle:96 (0 deg): RES-1.6K_1%_0402:264 ↔ RES-1.6K_1%_0402:265
- Angle:97 (0 deg): RES-1.6K_1%_0402:257 ↔ RES-1.6K_1%_0402:260
- Angle:98 (0 deg): RES-1.6K_1%_0402:260 ↔ RES-1.6K_1%_0402:261
- Angle:99 (0 deg): RES-1.6K_1%_0402:260 ↔ RES-1.6K_1%_0402:262
- [Flush]: RES-1.6K_1%_0402:266 ↔ RES-1.6K_1%_0402:267
- [Flush]: RES-1.6K_1%_0402:269 ↔ RES-1.6K_1%_0402:270
- [Flush]: RES-1.6K_1%_0402:268 ↔ RES-1.6K_1%_0402:269
- [Flush]: RES-1.6K_1%_0402:268 ↔ RES-1.6K_1%_0402:270
- [Angle] (0 deg): RES-1.6K_1%_0402:266 ↔ RES-1.6K_1%_0402:267
- [Angle] (0 deg): RES-1.6K_1%_0402:268 ↔ RES-1.6K_1%_0402:269
- [Angle] (0 deg): RES-1.6K_1%_0402:269 ↔ RES-1.6K_1%_0402:270
- Flush:515: RES-1.6K_1%_0402:259 ↔ RES-1.6K_1%_0402:268
- Flush:516: RES-1.6K_1%_0402:266 ↔ RES-1.6K_1%_0402:267
- Flush:517: RES-1.6K_1%_0402:263 ↔ RES-1.6K_1%_0402:267
- Flush:518: RES-1.6K_1%_0402:97 ↔ RES-1.6K_1%_0402:270
- [Flush]: RES-1.6K_1%_0402:274 ↔ RES-1.6K_1%_0402:275
- [Flush]: RES-1.6K_1%_0402:273 ↔ RES-1.6K_1%_0402:274
- [Flush]: RES-1.6K_1%_0402:273 ↔ RES-1.6K_1%_0402:275
- [Angle] (0 deg): RES-1.6K_1%_0402:273 ↔ RES-1.6K_1%_0402:274
- [Angle] (0 deg): RES-1.6K_1%_0402:274 ↔ RES-1.6K_1%_0402:275
- [Flush]: RES-1.6K_1%_0402:276 ↔ RES-1.6K_1%_0402:277
- [Flush]: RES-1.6K_1%_0402:279 ↔ RES-1.6K_1%_0402:280
- [Flush]: RES-1.6K_1%_0402:278 ↔ RES-1.6K_1%_0402:279
- [Flush]: RES-1.6K_1%_0402:278 ↔ RES-1.6K_1%_0402:280
- [Angle] (0 deg): RES-1.6K_1%_0402:276 ↔ RES-1.6K_1%_0402:277
- [Angle] (0 deg): RES-1.6K_1%_0402:278 ↔ RES-1.6K_1%_0402:279
- [Angle] (0 deg): RES-1.6K_1%_0402:279 ↔ RES-1.6K_1%_0402:280
- [Flush]: RES-1.6K_1%_0402:272 ↔ RES-1.6K_1%_0402:278
- [Flush]: RES-1.6K_1%_0402:276 ↔ RES-1.6K_1%_0402:277
- [Flush]: RES-1.6K_1%_0402:273 ↔ RES-1.6K_1%_0402:277
- Flush:530: RES-1.6K_1%_0402:277 ↔ RES-1.6K_1%_0402:278
- Flush:532: RES-1.6K_1%_0402:272 ↔ RES-1.6K_1%_0402:273
- Flush:533: RES-1.6K_1%_0402:275 ↔ RES-1.6K_1%_0402:278
- Flush:534: RES-1.6K_1%_0402:272 ↔ RES-1.6K_1%_0402:273
- Flush:535: RES-1.6K_1%_0402:263 ↔ RES-1.6K_1%_0402:268
- Mate:158: hw_LM - PCB:1 ↔ PESD2CANFD27V-UX:2
- Angle:109 (0 deg): STPS5H100AFY:3 ↔ PESD2CANFD27V-UX:2
- Flush:536: PESD2CANFD27V-UX:2 ↔ PESD2CANFD27V-UX:3
- Angle:110 (0 deg): KAM55CR72A106KV-C2220K-simpl:2 ↔ PESD2CANFD27V-UX:3
- [Flush]: RES-1.6K_1%_0402:285 ↔ RES-1.6K_1%_0402:286
- [Flush]: RES-1.6K_1%_0402:284 ↔ RES-1.6K_1%_0402:285
- [Flush]: RES-1.6K_1%_0402:284 ↔ RES-1.6K_1%_0402:286
- [Angle] (0 deg): RES-1.6K_1%_0402:284 ↔ RES-1.6K_1%_0402:285
- [Angle] (0 deg): RES-1.6K_1%_0402:285 ↔ RES-1.6K_1%_0402:286
- [Flush]: RES-1.6K_1%_0402:288 ↔ RES-1.6K_1%_0402:289
- [Flush]: RES-1.6K_1%_0402:287 ↔ RES-1.6K_1%_0402:288
- [Flush]: RES-1.6K_1%_0402:287 ↔ RES-1.6K_1%_0402:289
- [Angle] (0 deg): RES-1.6K_1%_0402:287 ↔ RES-1.6K_1%_0402:288
- [Angle] (0 deg): RES-1.6K_1%_0402:288 ↔ RES-1.6K_1%_0402:289
- [Flush]: RES-1.6K_1%_0402:286 ↔ RES-1.6K_1%_0402:287
- Flush:545: RES-1.6K_1%_0402:283 ↔ RES-1.6K_1%_0402:286
- Flush:546: RES-1.6K_1%_0402:280 ↔ RES-1.6K_1%_0402:283
- Flush:547: RES-1.6K_1%_0402:285 ↔ RES-1.6K_1%_0402:286
- Flush:548: RES-1.6K_1%_0402:286 ↔ RES-1.6K_1%_0402:289
- Flush:549: RES-1.6K_1%_0402:282 ↔ RES-1.6K_1%_0402:287
- Flush:550: RES-1.6K_1%_0402:258 ↔ RES-1.6K_1%_0402:283
- Flush:551: RES-1.6K_1%_0402:258 ↔ RES-1.6K_1%_0402:287
- [Flush]: RES-1.6K_1%_0402:290 ↔ RES-1.6K_1%_0402:291
- [Angle] (0 deg): RES-1.6K_1%_0402:290 ↔ RES-1.6K_1%_0402:291
- [Flush]: RES-1.6K_1%_0402:294 ↔ RES-1.6K_1%_0402:295
- [Flush]: RES-1.6K_1%_0402:293 ↔ RES-1.6K_1%_0402:294
- [Flush]: RES-1.6K_1%_0402:293 ↔ RES-1.6K_1%_0402:295
- [Angle] (0 deg): RES-1.6K_1%_0402:293 ↔ RES-1.6K_1%_0402:294
- [Angle] (0 deg): RES-1.6K_1%_0402:294 ↔ RES-1.6K_1%_0402:295
- [Flush]: RES-1.6K_1%_0402:297 ↔ RES-1.6K_1%_0402:298
- [Flush]: RES-1.6K_1%_0402:296 ↔ RES-1.6K_1%_0402:297
- [Flush]: RES-1.6K_1%_0402:296 ↔ RES-1.6K_1%_0402:298
- [Angle] (0 deg): RES-1.6K_1%_0402:296 ↔ RES-1.6K_1%_0402:297
- [Angle] (0 deg): RES-1.6K_1%_0402:297 ↔ RES-1.6K_1%_0402:298
- [Flush]: RES-1.6K_1%_0402:295 ↔ RES-1.6K_1%_0402:296
- [Flush]: RES-1.6K_1%_0402:292 ↔ RES-1.6K_1%_0402:295
- [Flush]: RES-1.6K_1%_0402:294 ↔ RES-1.6K_1%_0402:295
- [Flush]: RES-1.6K_1%_0402:295 ↔ RES-1.6K_1%_0402:298
- [Flush]: RES-1.6K_1%_0402:291 ↔ RES-1.6K_1%_0402:296
- Flush:564: RES-1.6K_1%_0402:282 ↔ RES-1.6K_1%_0402:297
- Flush:565: RES-1.6K_1%_0402:282 ↔ RES-1.6K_1%_0402:290
- Flush:566: RES-1.6K_1%_0402:289 ↔ RES-1.6K_1%_0402:291
- Flush:567: RES-1.6K_1%_0402:286 ↔ RES-1.6K_1%_0402:293
- [Flush]: RES-1.6K_1%_0402:301 ↔ RES-1.6K_1%_0402:302
- [Angle] (0 deg): RES-1.6K_1%_0402:301 ↔ RES-1.6K_1%_0402:302
- [Angle] (0 deg): RES-1.6K_1%_0402:299 ↔ RES-1.6K_1%_0402:300
- Flush:570: RES-1.6K_1%_0402:287 ↔ RES-1.6K_1%_0402:300
- Flush:571: RES-1.6K_1%_0402:283 ↔ RES-1.6K_1%_0402:299
- [Flush]: RES-1.6K_1%_0402:305 ↔ RES-1.6K_1%_0402:306
- [Angle] (0 deg): RES-1.6K_1%_0402:305 ↔ RES-1.6K_1%_0402:306
- [Angle] (0 deg): RES-1.6K_1%_0402:303 ↔ RES-1.6K_1%_0402:304
- [Flush]: RES-1.6K_1%_0402:309 ↔ RES-1.6K_1%_0402:310
- [Angle] (0 deg): RES-1.6K_1%_0402:309 ↔ RES-1.6K_1%_0402:310
- [Angle] (0 deg): RES-1.6K_1%_0402:307 ↔ RES-1.6K_1%_0402:308
- [Flush]: RES-1.6K_1%_0402:303 ↔ RES-1.6K_1%_0402:310
- [Flush]: RES-1.6K_1%_0402:305 ↔ RES-1.6K_1%_0402:308
- [Flush]: RES-1.6K_1%_0402:304 ↔ RES-1.6K_1%_0402:307
- Flush:577: RES-1.6K_1%_0402:301 ↔ RES-1.6K_1%_0402:304
- Flush:578: RES-1.6K_1%_0402:299 ↔ RES-1.6K_1%_0402:305
- Flush:579: RES-1.6K_1%_0402:288 ↔ RES-1.6K_1%_0402:307
- Flush:580: RES-1.6K_1%_0402:303 ↔ RES-1.6K_1%_0402:310
- [Flush]: RES-1.6K_1%_0402:313 ↔ RES-1.6K_1%_0402:314
- [Angle] (0 deg): RES-1.6K_1%_0402:313 ↔ RES-1.6K_1%_0402:314
- [Angle] (0 deg): RES-1.6K_1%_0402:311 ↔ RES-1.6K_1%_0402:312
- Flush:582: RES-1.6K_1%_0402:306 ↔ RES-1.6K_1%_0402:314
- Flush:583: RES-1.6K_1%_0402:288 ↔ RES-1.6K_1%_0402:312
- Flush:584: RES-1.6K_1%_0402:283 ↔ RES-1.6K_1%_0402:313
- Flush:585: RES-1.6K_1%_0402:306 ↔ RES-1.6K_1%_0402:311
- [Flush]: RES-1.6K_1%_0402:318 ↔ RES-1.6K_1%_0402:319
- [Angle] (0 deg): RES-1.6K_1%_0402:318 ↔ RES-1.6K_1%_0402:319
- [Angle] (0 deg): RES-1.6K_1%_0402:316 ↔ RES-1.6K_1%_0402:317
- Flush:588: RES-1.6K_1%_0402:288 ↔ RES-1.6K_1%_0402:317
- Flush:589: RES-1.6K_1%_0402:283 ↔ RES-1.6K_1%_0402:318
- Flush:590: RES-1.6K_1%_0402:306 ↔ RES-1.6K_1%_0402:321
- Flush:591: RES-1.6K_1%_0402:322 ↔ RES-1.6K_1%_0402:324
- Flush:592: RES-1.6K_1%_0402:322 ↔ RES-1.6K_1%_0402:323
- Flush:593: RES-1.6K_1%_0402:321 ↔ RES-1.6K_1%_0402:324
- Angle:134 (180 deg): hw_LM - PCB:1 ↔ AQ05C-01FTG:1
- Angle:135 (0 deg): hw_LM - PCB:1 ↔ AQ05C-01FTG:1
- Mate:159: hw_LM - PCB:1 ↔ AQ05C-01FTG:1
- Mate:163 (6.7 mm): hw_LM - PCB:1 ↔ P3767-pcba-envelop_20230310:1
- Mate:164: P3767-pcba-envelop_20230310:1 ↔ 9774065151:1
- Mate:165: hw_LM - PCB:1 ↔ 9774065151:1
- Mate:166: P3767-pcba-envelop_20230310:1 ↔ 9774065151:2
- Mate:167: hw_LM - PCB:1 ↔ 9774065151:2
- Mate:168: P3767-pcba-envelop_20230310:1 ↔ ATS-NVP-3281-C2-R0:1
- Mate:169: P3767-pcba-envelop_20230310:1 ↔ ATS-NVP-3281-C2-R0:1
- Mate:170: P3767-pcba-envelop_20230310:1 ↔ ATS-NVP-3281-C2-R0:1
- Mate:171: P3767-pcba-envelop_20230310:1 ↔ ATS-NVP-3281-C2-R0:1
- Flush:594: RES-1.6K_1%_0402:291 ↔ RES-1.6K_1%_0402:309
- Flush:595: RES-1.6K_1%_0402:225 ↔ RES-1.6K_1%_0402:262
- Flush:596: RES-1.6K_1%_0402:311 ↔ RES-1.6K_1%_0402:316
- Flush:597: RES-1.6K_1%_0402:312 ↔ RES-1.6K_1%_0402:315
- Mate:182: hw_LM - PCB:1 ↔ AUAV-L10D-M25125-RR-N:1
- Mate:184: hw_LM - PCB:1 ↔ SARA:1
- Mate:185: hw_LM - PCB:1 ↔ u-blox ZED-F9P:1
- Flush:601: DMN2710UTQ-7:6 ↔ DMN2710UTQ-7:9
- Flush:602: SN74LVC1G08QDCKRQ1:1 ↔ SN74LVC1G08QDCKRQ1:2
- Flush:603: DMN2710UTQ-7:7 ↔ DMN2710UTQ-7:10
- Mate:186: hw_LM - PCB:1 ↔ RESC-1210:1
- Angle:137 (0 deg): u-blox ZED-F9P:1 ↔ RESC-1210:1
- Mate:187: hw_LM - PCB:1 ↔ LTC7103MPUHE#PBF:1
- Angle:138 (0 deg): SARA:1 ↔ LTC7103MPUHE#PBF:1
- Mate:188: hw_LM - PCB:1 ↔ XAL4020-601MEC:3
- Mate:189: hw_LM - PCB:1 ↔ C1210C472KGRACAUTO:14
- Angle:139 (-90 deg): AUAV-L10D-M25125-RR-N:1 ↔ C1210C472KGRACAUTO:14
- Flush:604: C1210C472KGRACAUTO:15 ↔ C1210C472KGRACAUTO:16
- Flush:605: C1210C472KGRACAUTO:14 ↔ C1210C472KGRACAUTO:15
- Flush:606: C1210C472KGRACAUTO:16 ↔ C1210C472KGRACAUTO:17
- Flush:607: C1210C472KGRACAUTO:16 ↔ C1210C472KGRACAUTO:18
- Flush:608: C1210C472KGRACAUTO:15 ↔ C1210C472KGRACAUTO:17
- Flush:609: C1210C472KGRACAUTO:14 ↔ C1210C472KGRACAUTO:21
- Flush:610: C1210C472KGRACAUTO:20 ↔ C1210C472KGRACAUTO:21
- Mate:190 (0.1 mm): hw_LM - PCB:1 ↔ Body:1
- Mate:191: hw_LM - PCB:1 ↔ LPA-C011301S:1
- Flush:611: SML-D12V8WT86C:2 ↔ SML-D12V8WT86C:7
- Mate:192: hw_LM - PCB:1 ↔ MS561101BA03-50:1
- Angle:140 (0 deg): MS561101BA03-50:1 ↔ RES-1.6K_1%_0402:290
- Mate:193: hw_LM - PCB:1 ↔ DPS368XTSA1:1